# Autodesk Inventor assembly: s-assy-ring_gear-j2
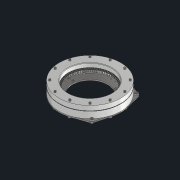
[picture p0: Inventor's stored thumbnail of the model, 180x180]
Saved by Autodesk Inventor 2022 (Build 260153000, 153)
## iProperties
Created: 2021-07-12
Part Number: s-assy-ring_gear-j2
Document SubType Name: Assembly
Designer: yuta0
Mass: 180.782 g
Surface Area: 832.349 cm^2
Volume: 122.833 cm^3
Density: 1.47176 g/cm^3
Author: yuta0
## Documents named in this file (11)
- C:\Users\yuta0\Documents\GitHub\catchrobo_hardware\assy-robot\s-assy-ring_gear-j2.iam
- C:\Users\yuta0\Documents\GitHub\catchrobo_hardware\assy-robot\base33.ipt
- C:\Users\yuta0\Documents\GitHub\catchrobo_hardware\assy-robot\carbon_plate13.ipt
- C:\Users\yuta0\Documents\GitHub\catchrobo_hardware\assy-robot\CB4-30.ipt
- C:\Users\yuta0\Documents\GitHub\catchrobo_hardware\assy-robot\base26.ipt
- C:\Users\yuta0\Documents\GitHub\catchrobo_hardware\assy-robot\SS-5GL.iam
- C:\Users\yuta0\Documents\GitHub\catchrobo_hardware\assy-robot\CB2-10.ipt
- C:\Users\yuta0\Documents\GitHub\catchrobo_hardware\assy-robot\LBNR2.ipt
- C:\Users\yuta0\Documents\GitHub\catchrobo_hardware\assy-robot\CBSTSR4-14.ipt
- C:\Users\yuta0\Documents\GitHub\catchrobo_hardware\assy-robot\CB4-6.ipt
- C:\Users\yuta0\Documents\GitHub\catchrobo_hardware\assy-robot\steel_plate6.ipt
## Components (25 placed, 10 different names)
1. base33:1 — フラッシュ:2, メイト:5, メイト:6, メイト:11, メイト:29, メイト:41
2. base26:1 — メイト:11, メイト:12, メイト:31
3. carbon_plate13:1 — メイト:4, メイト:5, メイト:6, メイト:12
4. steel_plate6:1 — メイト:30, メイト:32, メイト:40, メイト:41, メイト:48, 角度:52, メイト:49, メイト:50, メイト:51, メイト:52, メイト:53, メイト:54, メイト:55, メイト:56, メイト:57, メイト:58
5. SS-5GL:2 [sub-assembly] — メイト:40, メイト:45, メイト:57, メイト:58, メイト:59
6. CBSTSR4-14:1 — メイト:49, メイト:50
7. CBSTSR4-14:2 — メイト:51, メイト:52
8. CB4-6:1 — メイト:53, メイト:54
9. CB4-6:2 — メイト:55, メイト:56
10. CB4-30:1 — メイト:29, メイト:30
11. CB4-30:2
12. CB4-30:3
13. CB4-30:4
14. CB4-30:5
15. CB4-30:6
16. CB4-30:7
17. CB4-30:8
18. CB4-30:9
19. CB4-30:10
20. CB4-30:11
21. CB4-30:12
22. CB2-10:1 — メイト:45, メイト:59
23. LBNR2:1 — メイト:48
24. CB2-10:2
25. LBNR2:2
## Component patterns: (12 elements, first: CB4-30:1), (2 elements, first: CB2-10:1 + LBNR2:1)
## Relationships (26: Mate 24, Flush 1, Angle 1)
- フラッシュ:2 [Flush]: base33:1
- メイト:4 [Mate]: carbon_plate13:1
- メイト:5 [Mate]: base33:1 ↔ carbon_plate13:1
- メイト:6 [Mate]: base33:1 ↔ carbon_plate13:1
- メイト:11 [Mate]: base33:1 ↔ base26:1
- メイト:12 [Mate]: base26:1 ↔ carbon_plate13:1
- メイト:29 [Mate]: base33:1 ↔ CB4-30:1
- メイト:30 [Mate]: steel_plate6:1 ↔ CB4-30:1
- メイト:31 [Mate]: base26:1
- メイト:32 [Mate]: steel_plate6:1
- メイト:40 [Mate]: steel_plate6:1 ↔ SS-5GL:2
- メイト:41 [Mate]: base33:1 ↔ steel_plate6:1
- メイト:45 [Mate]: SS-5GL:2 ↔ CB2-10:1
- メイト:48 [Mate]: steel_plate6:1 ↔ LBNR2:1
- 角度:52 [Angle] (270 deg): steel_plate6:1
- メイト:49 [Mate]: steel_plate6:1 ↔ CBSTSR4-14:1
- メイト:50 [Mate]: steel_plate6:1 ↔ CBSTSR4-14:1
- メイト:51 [Mate]: steel_plate6:1 ↔ CBSTSR4-14:2
- メイト:52 [Mate]: steel_plate6:1 ↔ CBSTSR4-14:2
- メイト:53 [Mate]: steel_plate6:1 ↔ CB4-6:1
- メイト:54 [Mate]: steel_plate6:1 ↔ CB4-6:1
- メイト:55 [Mate]: steel_plate6:1 ↔ CB4-6:2
- メイト:56 [Mate]: steel_plate6:1 ↔ CB4-6:2
- メイト:57 [Mate]: steel_plate6:1 ↔ SS-5GL:2
- メイト:58 [Mate]: steel_plate6:1 ↔ SS-5GL:2
- メイト:59 [Mate]: SS-5GL:2 ↔ CB2-10:1
